# Autodesk Inventor assembly: ThArLampEnclosure
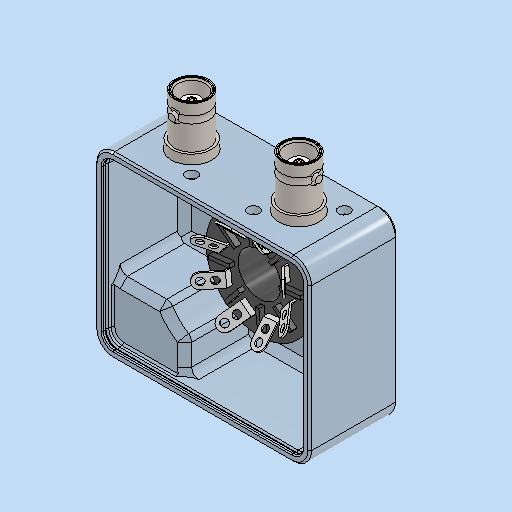
[picture p0: Inventor's stored thumbnail of the model, 512x512]
Saved by Autodesk Inventor 2025 (Build 290162000, 162)
## iProperties
Created: 2025-03-14
Part Number: ThArLampEnclosure
Document SubType Name: Assembly
Designer: kuzmin
Author: kuzmin
## Documents named in this file (5)
- C:\Users\queez\Dropbox\Drawings\PIHTI\ElectricAdapters\PL08\ThArLampEnclosure.iam
- C:\Users\queez\Dropbox\Drawings\PIHTI\ElectricAdapters\PL08\LampConnectorEnclosure.ipt
- C:\Users\queez\Dropbox\Drawings\PIHTI\ElectricAdapters\PL08\PL08.ipt
- C:\Users\queez\Dropbox\Drawings\PIHTI\ContentCenter\Electrics\Amphenol RF 31-203-RFX v1\Amphenol RF 31-203-RFX v1.ipt
- C:\Users\queez\Dropbox\Drawings\PIHTI\ElectricAdapters\PL08\LampConnectorEnclosure-lid.ipt
## Components (5 placed, 4 different names)
1. LampConnectorEnclosure:1 — Mate:1, Mate:2, Rigid:1, Rigid:2, Flush:1, Flush:2, Rigid:3
2. PL08:1 — Mate:1, Mate:2
3. Amphenol RF 31-203-RFX v1:1 — Rigid:1
4. Amphenol RF 31-203-RFX v1:2 — Rigid:2
5. LampConnectorEnclosure-lid:1 — Rigid:3
## Relationships (7: WeldJoint 3, Mate 2, Flush 2)
- Mate:1: LampConnectorEnclosure:1 ↔ PL08:1
- Mate:2: LampConnectorEnclosure:1 ↔ PL08:1
- Rigid:1 [WeldJoint]: LampConnectorEnclosure:1 ↔ Amphenol RF 31-203-RFX v1:1
- Rigid:2 [WeldJoint]: LampConnectorEnclosure:1 ↔ Amphenol RF 31-203-RFX v1:2
- Flush:1: LampConnectorEnclosure:1
- Flush:2: LampConnectorEnclosure:1
- Rigid:3 [WeldJoint]: LampConnectorEnclosure:1 ↔ LampConnectorEnclosure-lid:1
